# Autodesk Inventor assembly: Loop Assembly
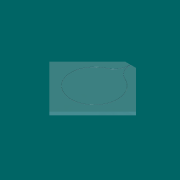
[picture p0: Inventor's stored thumbnail of the model, 180x180]
Saved by Autodesk Inventor 2020 (Build 240168000, 168)
## iProperties
Created: 2015-08-17
Part Number: Loop Assembly
Document SubType Name: Assembly
Designer: Cosmic
RuleStatus: InUse
Author: Cosmic
## Documents named in this file (5)
- C:\Users\sawaiz\oneDrive\projects\physics\muonTelescope\scintillatorPanel\loopPanel.iam
- C:\Users\sawaiz\oneDrive\projects\physics\muonTelescope\scintillatorPanel\loopPanel.ipt
- C:\Users\sawaiz\oneDrive\projects\physics\muonTelescope\scintillatorPanel\fiberLoop.ipt
- C:\Users\sawaiz\OneDrive\projects\physics\muonTelescope\scintillatorPanel\opticalCement.ipt
- C:\Users\sawaiz\oneDrive\projects\physics\muonTelescope\scintillatorPanel\Scintillator.xlsx
## Components (3 placed, 3 different names)
1. loopPanel:1 — Mate:1, Mate:2, Flush:1, Mate:3, Mate:4, Flush:2
2. fiberLoop:1 — Mate:1, Mate:2, Flush:1
3. opticalCement:1 — Mate:3, Mate:4, Flush:2
## Relationships (6: Mate 4, Flush 2)
- Mate:1: loopPanel:1 ↔ fiberLoop:1
- Mate:2: loopPanel:1 ↔ fiberLoop:1
- Flush:1: loopPanel:1 ↔ fiberLoop:1
- Mate:3: loopPanel:1 ↔ opticalCement:1
- Mate:4: loopPanel:1 ↔ opticalCement:1
- Flush:2: loopPanel:1 ↔ opticalCement:1
## Named parameters: OpticalFiberClearence = 0.15 mm, MPPCClearence = 0.075 mm, FiberSensorClerence = 0.5 mm, OpticalFiberDiameter = 1 mm, ScintillatorThickness = 10 mm, SmallTrackDiameter = 175 mm, LargeTrackRatio = 3, ScintillatorEdgeClearence = 3 mm, ScintillatorWidth = 200 mm, ScintillatorHeight = 200 mm, ShallowTrackDepth = 1.3 mm, MPPCSensorClearence = 1.45 mm, MPPCSensorOffsett = 2.105 mm, MPPCWidth = 5.9 mm, MPPCHeight = 6.55 mm, FiberEdgeOffsett = 5 mm, MPPCDepth = 1 mm, LongFiberAngle = 30 deg, ShortFiberAngle = 78 deg, LoopLargeTrackRatio = 1.5, LoopSmallTrackDiameter = 100 mm, MountingScrewDepth = 4 mm, MountingScrewOffsett = 20 mm, LoopLength = 150 mm, cornerChamfer = 25.4 mm, mountingSpacing = 18 mm, rubberizedCoating = 0.0508, silveringThickness = 0.2 mm
note: some values were not read from the file. Shown as the stored number, unit unknown: "rubberizedCoating".
